# Autodesk Inventor assembly: acrylic_assemble
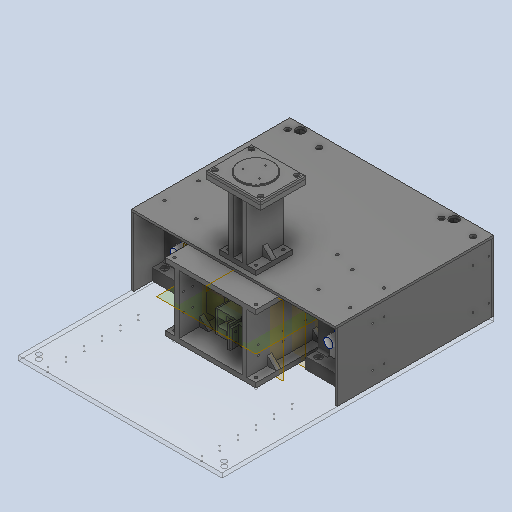
[picture p0: Inventor's stored thumbnail of the model, 512x512]
Saved by Autodesk Inventor 2026.2 (Build 302298010, 298A)
## iProperties
Created: 2026-05-13
Part Number: acrylic_assemble
Document SubType Name: Assembly
Designer: chris
Author: chris
## Documents named in this file (13)
- C:\Users\chanh\내 드라이브\교과공부\2026년 1학기 (4학년 1학기)\01창의제품설계\UMMA_CAD\04그리퍼\acrilic\acrylic_assemble.iam
- C:\Users\chanh\내 드라이브\교과공부\2026년 1학기 (4학년 1학기)\01창의제품설계\UMMA_CAD\04그리퍼\acrilic\acrylic.ipt
- C:\Users\chanh\내 드라이브\교과공부\2026년 1학기 (4학년 1학기)\01창의제품설계\UMMA_CAD\04그리퍼\acrilic\actuator_bracket\test3_hw.ipt
- C:\Users\chanh\내 드라이브\교과공부\2026년 1학기 (4학년 1학기)\01창의제품설계\UMMA_CAD\04그리퍼\acrilic\actuator_bracket\test2_hw.ipt
- C:\Users\chanh\내 드라이브\교과공부\2026년 1학기 (4학년 1학기)\01창의제품설계\UMMA_CAD\04그리퍼\acrilic\actuator_bracket\test4_hw.ipt
- C:\Users\chanh\내 드라이브\교과공부\2026년 1학기 (4학년 1학기)\01창의제품설계\UMMA_CAD\04그리퍼\acrilic\case\case.iam
- C:\Users\chanh\내 드라이브\교과공부\2026년 1학기 (4학년 1학기)\01창의제품설계\UMMA_CAD\04그리퍼\acrilic\acrylic_upper.ipt
- C:\Users\chanh\내 드라이브\교과공부\2026년 1학기 (4학년 1학기)\01창의제품설계\UMMA_CAD\04그리퍼\acrilic\acrylic_back.ipt
- C:\Users\chanh\내 드라이브\교과공부\2026년 1학기 (4학년 1학기)\01창의제품설계\UMMA_CAD\04그리퍼\acrilic\acrylic_side.ipt
- C:\Users\chanh\내 드라이브\교과공부\2026년 1학기 (4학년 1학기)\01창의제품설계\UMMA_CAD\04그리퍼\acrilic\lidar\lidar.ipt
- C:\Users\chanh\내 드라이브\교과공부\2026년 1학기 (4학년 1학기)\01창의제품설계\UMMA_CAD\04그리퍼\acrilic\lidar\LiDAR_holder_upper.ipt
- C:\Users\chanh\내 드라이브\교과공부\2026년 1학기 (4학년 1학기)\01창의제품설계\UMMA_CAD\04그리퍼\acrilic\actuator_bracket\Linear Motor (T-Frame).ipt
- C:\Users\chanh\내 드라이브\교과공부\2026년 1학기 (4학년 1학기)\01창의제품설계\UMMA_CAD\04그리퍼\acrilic\actuator_bracket\Linear Motor Bar (T-Frame).ipt
## Components (18 placed, 12 different names)
1. acrylic:1 — Flush:1, Flush:2, Flush:3, Mate:1, Insert:1, Mate:2, Insert:2, Mate:3, Insert:3, Insert:4, Insert:5, Insert:6, Mate:4, Flush:4, Flush:5, Flush:6, Mate:5, Flush:7, Flush:8, Mate:6, Flush:9, Insert:7, Insert:8, Insert:9, Insert:10, Insert:11, Flush:10, Flush:11, Mate:7, Mate:9, Mate:12
2. test3_hw:1 — Mate:1, Insert:1, Mate:8, Flush:12
3. test2_hw:1 — Mate:2, Insert:2
4. test4_hw:1 — Mate:3, Insert:3, Insert:4
5. case:1 [sub-assembly] — Insert:5, Insert:6
6. acrylic_upper:1 — Mate:4, Flush:4, Flush:5, Insert:14, Insert:15
7. acrylic_back:1 — Flush:6, Mate:5, Flush:7
8. acrylic_side:1 — Flush:8, Mate:6, Flush:9
9. test3_hw:2 — Insert:11, Mate:11, Flush:13
10. test2_hw:2 — Insert:7, Insert:8
11. test4_hw:2 — Insert:9, Insert:10
12. acrylic_side:2 — Flush:10, Flush:11, Mate:7
13. lidar:1 — Insert:12, Insert:13, Insert:14, Insert:15
14. LiDAR_holder_upper:1 — Insert:12, Insert:13
15. Linear Motor (T-Frame):1 — Mate:8, Flush:12, Mate:9, Mate:10, Insert:16
16. Linear Motor (T-Frame):2 — Mate:11, Flush:13, Mate:12, Insert:17
17. Linear Motor Bar (T-Frame):1 — Mate:10, Insert:16
18. Linear Motor Bar (T-Frame):2 — Insert:17
## Relationships (42: Insert 17, Flush 13, Mate 12)
- Flush:1: acrylic:1
- Flush:2: acrylic:1
- Flush:3: acrylic:1
- Mate:1: acrylic:1 ↔ test3_hw:1
- Insert:1: acrylic:1 ↔ test3_hw:1
- Mate:2: acrylic:1 ↔ test2_hw:1
- Insert:2: acrylic:1 ↔ test2_hw:1
- Mate:3: acrylic:1 ↔ test4_hw:1
- Insert:3: acrylic:1 ↔ test4_hw:1
- Insert:4: acrylic:1 ↔ test4_hw:1
- Insert:5: acrylic:1 ↔ case:1
- Insert:6: acrylic:1 ↔ case:1
- Mate:4 (150 mm): acrylic:1 ↔ acrylic_upper:1
- Flush:4: acrylic:1 ↔ acrylic_upper:1
- Flush:5: acrylic:1 ↔ acrylic_upper:1
- Flush:6: acrylic:1 ↔ acrylic_back:1
- Mate:5: acrylic:1 ↔ acrylic_back:1
- Flush:7: acrylic:1 ↔ acrylic_back:1
- Flush:8: acrylic:1 ↔ acrylic_side:1
- Mate:6: acrylic:1 ↔ acrylic_side:1
- Flush:9 (5 mm): acrylic:1 ↔ acrylic_side:1
- Insert:7: acrylic:1 ↔ test2_hw:2
- Insert:8: acrylic:1 ↔ test2_hw:2
- Insert:9: acrylic:1 ↔ test4_hw:2
- Insert:10: acrylic:1 ↔ test4_hw:2
- Insert:11: acrylic:1 ↔ test3_hw:2
- Flush:10: acrylic:1 ↔ acrylic_side:2
- Flush:11: acrylic:1 ↔ acrylic_side:2
- Mate:7: acrylic:1 ↔ acrylic_side:2
- Insert:12: lidar:1 ↔ LiDAR_holder_upper:1
- Insert:13: lidar:1 ↔ LiDAR_holder_upper:1
- Insert:14: acrylic_upper:1 ↔ lidar:1
- Insert:15: acrylic_upper:1 ↔ lidar:1
- Mate:8: test3_hw:1 ↔ Linear Motor (T-Frame):1
- Flush:12: test3_hw:1 ↔ Linear Motor (T-Frame):1
- Mate:9 (-55 mm): acrylic:1 ↔ Linear Motor (T-Frame):1
- Mate:10: Linear Motor (T-Frame):1 ↔ Linear Motor Bar (T-Frame):1
- Insert:16 (-222 mm): Linear Motor (T-Frame):1 ↔ Linear Motor Bar (T-Frame):1
- Mate:11: test3_hw:2 ↔ Linear Motor (T-Frame):2
- Flush:13: test3_hw:2 ↔ Linear Motor (T-Frame):2
- Mate:12 (-55 mm): acrylic:1 ↔ Linear Motor (T-Frame):2
- Insert:17 (-222 mm): Linear Motor (T-Frame):2 ↔ Linear Motor Bar (T-Frame):2
